# Autodesk Inventor assembly: RodaOmni 60 mm
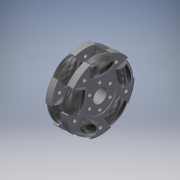
[picture p0: Inventor's stored thumbnail of the model, 180x180]
Saved by Autodesk Inventor 2017.3 (Build 213257000, 257)
## iProperties
Created: 2020-07-20
Part Number: RodaOmni 60 mm
Document SubType Name: Assembly
Designer: Fahar Endra
Author: Fahar Endra
## Documents named in this file (3)
- D:\Robotik KRSBI\Roda Omni 60 mm\RodaOmni 60 mm.iam
- D:\Robotik KRSBI\Roda Omni 60 mm\Dasar.ipt
- D:\Robotik KRSBI\Roda Omni 60 mm\Roller.ipt
## Components (12 placed, 2 different names)
1. Dasar:1 — Rotational:1, Rotational:2, Rotational:3, Rotational:4, Rotational:5, Rigid:1
2. Roller:1 — Rotational:1
3. Roller:2 — Rotational:2
4. Roller:3 — Rotational:4
5. Roller:4 — Rotational:5
6. Roller:5 — Rotational:3
7. Dasar:2 — Rigid:1, Rotational:6, Rotational:7, Rotational:8, Rotational:9, Rotational:10
8. Roller:6 — Rotational:8
9. Roller:7 — Rotational:6
10. Roller:8 — Rotational:9
11. Roller:9 — Rotational:7
12. Roller:10 — Rotational:10
## Relationships (11: RevoluteJoint 10, WeldJoint 1)
- Rotational:1 [RevoluteJoint]: Dasar:1 ↔ Roller:1
- Rotational:2 [RevoluteJoint]: Dasar:1 ↔ Roller:2
- Rotational:3 [RevoluteJoint]: Dasar:1 ↔ Roller:5
- Rotational:4 [RevoluteJoint]: Dasar:1 ↔ Roller:3
- Rotational:5 [RevoluteJoint]: Dasar:1 ↔ Roller:4
- Rigid:1 [WeldJoint]: Dasar:1 ↔ Dasar:2
- Rotational:6 [RevoluteJoint]: Dasar:2 ↔ Roller:7
- Rotational:7 [RevoluteJoint]: Dasar:2 ↔ Roller:9
- Rotational:8 [RevoluteJoint]: Dasar:2 ↔ Roller:6
- Rotational:9 [RevoluteJoint]: Dasar:2 ↔ Roller:8
- Rotational:10 [RevoluteJoint]: Dasar:2 ↔ Roller:10
